# Autodesk Inventor assembly: Tesis_Assembly
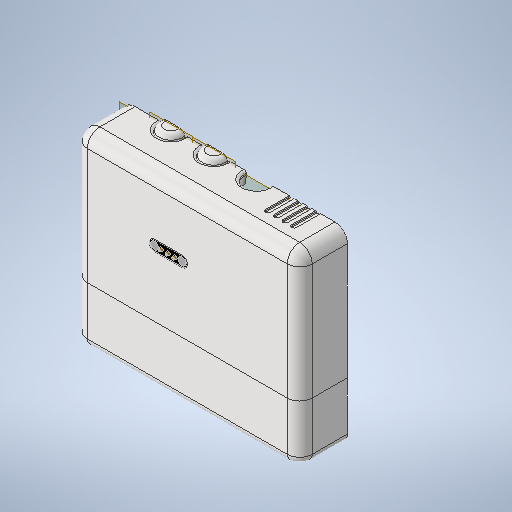
[picture p0: Inventor's stored thumbnail of the model, 512x512]
Saved by Autodesk Inventor 2025.1 (Build 291241000, 241)
## iProperties
Created: 2025-05-06
Part Number: Tesis_Assembly
Document SubType Name: Assembly
Designer: santiago
Author: santiago
## Documents named in this file (17)
- C:\Users\santiago\Documents\Tesis\3d models\Tesis_Assembly.iam
- C:\Users\santiago\Documents\Tesis\3d models\conn\2_pin_ear_female.ipt
- C:\Users\santiago\Documents\Tesis\3d models\conn\3_pin_ear_female.ipt
- C:\Users\santiago\Documents\Tesis\3d models\conn\3_pin_no_ear_male.ipt
- C:\Users\santiago\Documents\Tesis\3d models\conn\M3 x 10.ipt
- C:\Users\santiago\Documents\Tesis\3d models\conn\M3 x 16.ipt
- C:\Users\santiago\Documents\Tesis\3d models\conn\shell_bttm.ipt
- C:\Users\santiago\Documents\Tesis\3d models\conn\shell_top.ipt
- C:\Users\santiago\Documents\Tesis\3d models\Bottom_layer.iam
- C:\Users\santiago\Documents\Tesis\3d models\Top_layer.iam
- C:\Users\santiago\Documents\Tesis\3d models\scaled\cam.ipt
- C:\Users\santiago\Documents\Tesis\3d models\scaled\Electromagnet.ipt
- C:\Users\santiago\Documents\Tesis\3d models\scaled\CUSTOM\Part5.ipt
- C:\Users\santiago\Documents\Tesis\3d models\conn_enclosure.ipt
- C:\Users\santiago\Documents\Tesis\3d models\inner_bttm.ipt
- C:\Users\santiago\Documents\Tesis\3d models\inner_top.ipt
- C:\Users\santiago\Documents\Tesis\3d models\scaled\CUSTOM\custom_cam.ipt
## Components (26 placed, 16 different names)
1. 2_pin_ear_female:1 — Insert:15, Mate:13
2. 3_pin_ear_female:1 — Insert:20, Mate:14
3. 3_pin_no_ear_male:1
4. shell_bttm:1 — Insert:15, Mate:10, Flush:3, Mate:12, Insert:19, Mate:13
5. shell_top:1 — Mate:10, Flush:3, Mate:11, Insert:18, Mate:12, Insert:20, Mate:14
6. Bottom_layer:1 [sub-assembly] — Mate:7, Mate:8, Flush:2, Mate:15
7. Top_layer:1 [sub-assembly] — Mate:4, Mate:5, Mate:6, Mate:7, Mate:8, Flush:2
8. conn_enclosure:1 — Insert:7, Insert:8, Insert:16, Mate:11, Mate:15
9. inner_bttm:1 — Mate:3, Flush:1, Insert:4, Insert:5, Insert:6, Mate:4, Insert:7, Insert:8, Insert:21
10. inner_top:1 — Insert:5, Insert:6, Insert:18, Mate:16, Mate:17, Mate:18
11. cam:1 — Mate:3, Flush:1, Transitional:1
12. Part5:1 — Mate:16, Transitional:1, Mate:17
13. custom_cam:1 — Insert:21, Transitional:2
14. Part5:2 — Mate:18, Transitional:2
15. Electromagnet:1 — Insert:4, Mate:5
16. Electromagnet:2
17. Electromagnet:3
18. Electromagnet:4
19. Electromagnet:5 — Mate:6
20. Electromagnet:6
21. M3 x 10:1 — Insert:16
22. M3 x 10:2
23. M3 x 16:1 — Insert:19
24. M3 x 16:2
25. M3 x 16:3
26. M3 x 16:4
## Component patterns: (6 elements, first: Electromagnet:1), (2 elements, first: M3 x 10:1), (4 elements, first: M3 x 16:1)
## Relationships (31: Mate 15, Insert 11, Flush 3, Transitional 2)
- Mate:3: inner_bttm:1 ↔ cam:1
- Flush:1: inner_bttm:1 ↔ cam:1
- Insert:4 (-1.29 mm): inner_bttm:1 ↔ Electromagnet:1
- Insert:5: inner_bttm:1 ↔ inner_top:1
- Insert:6: inner_bttm:1 ↔ inner_top:1
- Mate:4: Top_layer:1 ↔ inner_bttm:1
- Mate:5: Top_layer:1 ↔ Electromagnet:1
- Mate:6: Top_layer:1 ↔ Electromagnet:5
- Mate:7: Bottom_layer:1 ↔ Top_layer:1
- Mate:8: Bottom_layer:1 ↔ Top_layer:1
- Flush:2: Bottom_layer:1 ↔ Top_layer:1
- Insert:7: conn_enclosure:1 ↔ inner_bttm:1
- Insert:8: conn_enclosure:1 ↔ inner_bttm:1
- Insert:15: 2_pin_ear_female:1 ↔ shell_bttm:1
- Insert:16: conn_enclosure:1 ↔ M3 x 10:1
- Mate:10: shell_bttm:1 ↔ shell_top:1
- Flush:3: shell_bttm:1 ↔ shell_top:1
- Mate:11: shell_top:1 ↔ conn_enclosure:1
- Insert:18: shell_top:1 ↔ inner_top:1
- Mate:12: shell_bttm:1 ↔ shell_top:1
- Insert:19: shell_bttm:1 ↔ M3 x 16:1
- Mate:13: 2_pin_ear_female:1 ↔ shell_bttm:1
- Insert:20: 3_pin_ear_female:1 ↔ shell_top:1
- Mate:14: 3_pin_ear_female:1 ↔ shell_top:1
- Mate:15: Bottom_layer:1 ↔ conn_enclosure:1
- Mate:16: inner_top:1 ↔ Part5:1
- Transitional:1: cam:1 ↔ Part5:1
- Mate:17: inner_top:1 ↔ Part5:1
- Insert:21: inner_bttm:1 ↔ custom_cam:1
- Mate:18: inner_top:1 ↔ Part5:2
- Transitional:2: custom_cam:1 ↔ Part5:2
## Named parameters: COLUMN = 60.8 mm
